# Autodesk Inventor assembly: WheelAssembly
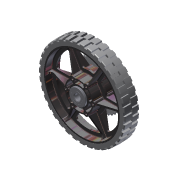
[picture p0: Inventor's stored thumbnail of the model, 180x180]
Saved by Autodesk Inventor 2012 (Build 160160000, 160)
## iProperties
Created: 2012-01-08
Part Number: WheelAssembly
Document SubType Name: Assembly
Designer: JesseK
Author: JesseK
## Documents named in this file (4)
- C:\Users\William\Dropbox\Robotics\CAD\team1885frc\Robot2012\DriveTrain\WheelAssembly.iam
- C:\Users\William\Dropbox\Robotics\CAD\team1885frc\AndyMark\HiGrip6in\6-HiGrip-am-0940.iam
- C:\Users\William\Dropbox\Robotics\CAD\team1885frc\Hardware\Sprockets\FlatSprocket_Num25_40T_0.875bore.ipt
- C:\Users\William\Dropbox\Robotics\CAD\team1885frc\Hardware\Bolts\ThreadForming_Num10_24_0.75len_HexHead.ipt
## Components (8 placed, 3 different names)
1. 6-HiGrip-am-0940:1 [sub-assembly] — Mate:13, Mate:14, Mate:15
2. FlatSprocket_Num25_40T_0.875bore:1 — Mate:1, Mate:2, Mate:3, Mate:4, Mate:5, Mate:6, Mate:7, Mate:8, Mate:9, Mate:10, Mate:11, Mate:12, Mate:13
3. ThreadForming_Num10_24_0.75len_HexHead:1 — Mate:1, Mate:8, Mate:15
4. ThreadForming_Num10_24_0.75len_HexHead:2 — Mate:2, Mate:7, Mate:14
5. ThreadForming_Num10_24_0.75len_HexHead:3 — Mate:3, Mate:9
6. ThreadForming_Num10_24_0.75len_HexHead:4 — Mate:4, Mate:10
7. ThreadForming_Num10_24_0.75len_HexHead:5 — Mate:5, Mate:11
8. ThreadForming_Num10_24_0.75len_HexHead:6 — Mate:6, Mate:12
## Relationships (15: Mate 15)
- Mate:1: FlatSprocket_Num25_40T_0.875bore:1 ↔ ThreadForming_Num10_24_0.75len_HexHead:1
- Mate:2: FlatSprocket_Num25_40T_0.875bore:1 ↔ ThreadForming_Num10_24_0.75len_HexHead:2
- Mate:3: FlatSprocket_Num25_40T_0.875bore:1 ↔ ThreadForming_Num10_24_0.75len_HexHead:3
- Mate:4: FlatSprocket_Num25_40T_0.875bore:1 ↔ ThreadForming_Num10_24_0.75len_HexHead:4
- Mate:5: FlatSprocket_Num25_40T_0.875bore:1 ↔ ThreadForming_Num10_24_0.75len_HexHead:5
- Mate:6: FlatSprocket_Num25_40T_0.875bore:1 ↔ ThreadForming_Num10_24_0.75len_HexHead:6
- Mate:7: FlatSprocket_Num25_40T_0.875bore:1 ↔ ThreadForming_Num10_24_0.75len_HexHead:2
- Mate:8: FlatSprocket_Num25_40T_0.875bore:1 ↔ ThreadForming_Num10_24_0.75len_HexHead:1
- Mate:9: FlatSprocket_Num25_40T_0.875bore:1 ↔ ThreadForming_Num10_24_0.75len_HexHead:3
- Mate:10: FlatSprocket_Num25_40T_0.875bore:1 ↔ ThreadForming_Num10_24_0.75len_HexHead:4
- Mate:11: FlatSprocket_Num25_40T_0.875bore:1 ↔ ThreadForming_Num10_24_0.75len_HexHead:5
- Mate:12: FlatSprocket_Num25_40T_0.875bore:1 ↔ ThreadForming_Num10_24_0.75len_HexHead:6
- Mate:13: 6-HiGrip-am-0940:1 ↔ FlatSprocket_Num25_40T_0.875bore:1
- Mate:14: 6-HiGrip-am-0940:1 ↔ ThreadForming_Num10_24_0.75len_HexHead:2
- Mate:15: 6-HiGrip-am-0940:1 ↔ ThreadForming_Num10_24_0.75len_HexHead:1
